# Autodesk Inventor assembly: EV-ADF41020
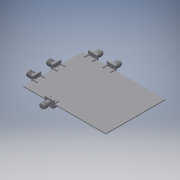
[picture p0: Inventor's stored thumbnail of the model, 180x180]
Saved by Autodesk Inventor 2018 (Build 220112000, 112)
## iProperties
Created: 2018-04-06
Part Number: EV-ADF41020
Document SubType Name: Assembly
Designer: bbramman
Author: bbramman
## Documents named in this file (3)
- C:\Users\bbramman\OneDrive\Documents\Trapped Ion Research (Grad)\Electronics\pll-evalboard-synthesizer\Box CAD\EV-ADF41020.iam
- C:\Users\bbramman\OneDrive\Documents\Trapped Ion Research (Grad)\Electronics\pll-evalboard-synthesizer\Box CAD\90x65mm-PCB.ipt
- C:\Users\bbramman\OneDrive\Documents\Trapped Ion Research (Grad)\Electronics\pll-evalboard-synthesizer\Box CAD\SMA-END.ipt
## Components (6 placed, 2 different names)
1. 90x65mm-PCB:1 — Mate:1, Mate:2, Mate:3, Mate:4, Mate:5, Mate:6, Mate:7, Mate:8, Mate:9, Mate:10
2. SMA-END:1 — Mate:5, Mate:7
3. SMA-END:2 — Mate:4, Mate:8
4. SMA-END:3 — Mate:3, Mate:6
5. SMA-END:4 — Mate:1, Mate:9
6. SMA-END:5 — Mate:2, Mate:10
## Relationships (10: Mate 10)
- Mate:1: 90x65mm-PCB:1 ↔ SMA-END:4
- Mate:2: 90x65mm-PCB:1 ↔ SMA-END:5
- Mate:3: 90x65mm-PCB:1 ↔ SMA-END:3
- Mate:4: 90x65mm-PCB:1 ↔ SMA-END:2
- Mate:5: 90x65mm-PCB:1 ↔ SMA-END:1
- Mate:6: 90x65mm-PCB:1 ↔ SMA-END:3
- Mate:7: 90x65mm-PCB:1 ↔ SMA-END:1
- Mate:8: 90x65mm-PCB:1 ↔ SMA-END:2
- Mate:9: 90x65mm-PCB:1 ↔ SMA-END:4
- Mate:10: 90x65mm-PCB:1 ↔ SMA-END:5
